# Autodesk Inventor assembly: Kepler Vibe Assembly
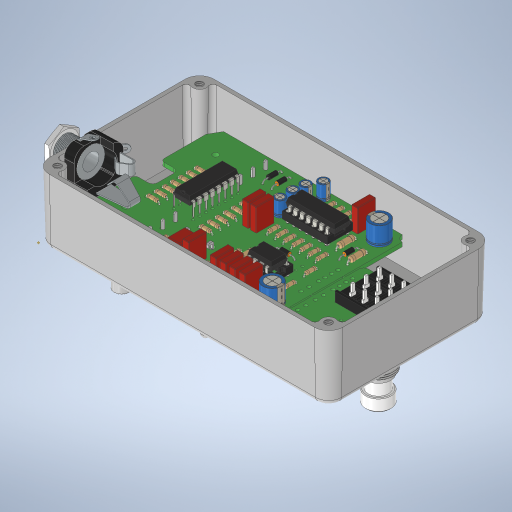
[picture p0: Inventor's stored thumbnail of the model, 512x512]
Saved by Autodesk Inventor 2023 (Build 270158030, 158C)
## iProperties
Created: 2022-11-10
Part Number: Kepler Vibe Assembly
Document SubType Name: Assembly
Designer: Imogen Heard
Author: Imogen Heard
## iProperties of the stored document Nut- M9x0.5mm^1~4in Mono Jack Socket.ipt
Created: 2013-10-17
Part Number: Nut- M9x0.5mm^1~4in Mono Jack Socket
Material: Generic
Document SubType Name: Modeling
Designer: Imogen Heard
Density: 1 g/cm^3
Appearance: Default
Author: Imogen Heard
Sending System: SolidWorks 2012
Last Author: htlr&d04
Last Saved: 2013-10-18
## iProperties of the stored document Copy of 1~4in Mono Jack Socket^1~4in Mono Jack Socket.ipt
Created: 2013-10-17
Part Number: Copy of 1~4in Mono Jack Socket^1~4in Mono Jack Socket
Material: Generic
Document SubType Name: Modeling
Designer: Imogen Heard
Density: 1 g/cm^3
Appearance: Default
Author: Imogen Heard
Sending System: SolidWorks 2012
Last Author: htlr&d04
Last Saved: 2013-10-18
## iProperties of the stored document 1~4in Mono Jack Socket.iam
Created: 2013-10-17
Part Number: 1~4in Mono Jack Socket
Document SubType Name: Assembly
Designer: Imogen Heard
Author: Imogen Heard
Sending System: SolidWorks 2012
Last Author: htlr&d04
Last Saved: 2013-10-18
## Documents named in this file (7)
- **C:\Users\dheard\Documents\Inventor\Inventor_Projects\Electronics Projects\Kepler Vibe Assembly.iam*LocalDocs*xAaaaqrdaAaaaaaaaAaaaqqgmMc*Nut- M9x0.5mm^1~4in Mono Jack Socket.ipt
- **C:\Users\dheard\Documents\Inventor\Inventor_Projects\Electronics Projects\Kepler Vibe Assembly.iam*LocalDocs*xAaaaapbaAaaaaaaaAaaaqditUh*Copy of 1~4in Mono Jack Socket^1~4in Mono Jack Socket.ipt
- **C:\Users\dheard\Documents\Inventor\Inventor_Projects\Electronics Projects\Kepler Vibe Assembly.iam*LocalDocs*xAaaaqubaAaaaaaaaAaaaqnddDg*1~4in Mono Jack Socket.iam
- C:\Users\dheard\Documents\Inventor\Inventor_Projects\Electronics Projects\Kepler Vibe Assembly.iam
- C:\Users\dheard\Documents\Inventor\Inventor_Projects\Electronics Projects\Kepler Vibe Enclosure.ipt
- C:\Users\dheard\Documents\Inventor\Inventor_Projects\Electronics Projects\Kepler_Vibe_PCB_v2.ipt
- C:\Users\dheard\Documents\0000.KiCad\6.0\3rdparty\000_Immo_3D_models\1-4-inch-mono-jack-socket-1.snapshot.2\Renderings\1~4in Mono Jack Socket.SLDASM
## Components (3 placed, 3 different names)
1. Kepler Vibe Enclosure:1 — Mate:1, Mate:2, Mate:3, Mate:4
2. Kepler_Vibe_PCB_v2:1 — Mate:1, Mate:2, Mate:3
3. 1~4in Mono Jack Socket:3 [sub-assembly] — Mate:4
## Relationships (4: Mate 4)
- Mate:1: Kepler Vibe Enclosure:1 ↔ Kepler_Vibe_PCB_v2:1
- Mate:2 (2 mm): Kepler Vibe Enclosure:1 ↔ Kepler_Vibe_PCB_v2:1
- Mate:3 (30 mm): Kepler Vibe Enclosure:1 ↔ Kepler_Vibe_PCB_v2:1
- Mate:4: Kepler Vibe Enclosure:1 ↔ 1~4in Mono Jack Socket:3
